# Autodesk Inventor assembly: emsamble caja
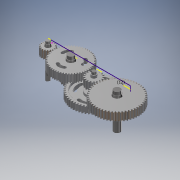
[picture p0: Inventor's stored thumbnail of the model, 180x180]
Saved by Autodesk Inventor 2018 (Build 220112000, 112)
## iProperties
Created: 2017-08-31
Part Number: emsamble caja
Material: Genérico
Document SubType Name: Assembly
Designer: Alumno
Author: Alumno
## Documents named in this file (14)
- D:\Documents\Desktop\proyecto caja reductora-II\emsamble caja.iam
- D:\Documents\Desktop\proyecto caja reductora-II\EJE 2 (30 mm y 15 mm).iam
- D:\Documents\Desktop\proyecto caja reductora-II\TREN 1\Design Accelerator\Engranaje recto12.ipt
- D:\Documents\Desktop\proyecto caja reductora-II\TREN 1\Design Accelerator\Engranaje recto22.ipt
- D:\Documents\Desktop\proyecto caja reductora-II\TREN 2\Design Accelerator\Engranaje recto11.ipt
- D:\Documents\Desktop\proyecto caja reductora-II\TREN 2\Design Accelerator\Engranaje recto21.ipt
- D:\Documents\Desktop\proyecto caja reductora-II\TREN 3\Design Accelerator\Engranaje recto11.ipt
- D:\Documents\Desktop\proyecto caja reductora-II\TREN 3\Design Accelerator\Engranaje recto21.ipt
- D:\Documents\Desktop\proyecto caja reductora-II\EJE 3 (30-45).iam
- D:\Documents\Desktop\proyecto caja reductora-II\EJE 4.iam
- D:\Documents\Desktop\proyecto caja reductora-II\Chaveta- Tren 1.ipt
- D:\Documents\Desktop\proyecto caja reductora-II\Chaveta 25.ipt
- D:\Documents\Desktop\proyecto caja reductora-II\EJE 1.iam
- D:\Documents\Desktop\proyecto caja reductora-II\RODAMIENTO 15 D\6002.iam
## Components (14 placed, 9 different names)
1. Engranaje recto1:1 — Coincidencia:1, Ángulo:2, Coincidencia:16
2. Engranaje recto2:1 — Coincidencia:5, Coincidencia:6, Ángulo:2, Coincidencia:17
3. Engranaje recto2:2 — Coincidencia:12, Coincidencia:13, Coincidencia:18
4. Engranaje recto1:3 — Coincidencia:14, Coincidencia:15
5. Engranaje recto2:3 — Coincidencia:22, Coincidencia:23, Coincidencia:24
6. EJE 2 (30 mm y 15 mm):3 [sub-assembly] — Coincidencia:2, Coincidencia:3, Coincidencia:4, Coincidencia:5, Ángulo:1, Ángulo:3, Coincidencia:17, Nivelación:1, Coincidencia:25, Coincidencia:26
7. Engranaje recto1:4 — Coincidencia:25, Coincidencia:26
8. EJE 3 (30-45):1 [sub-assembly] — Coincidencia:9, Coincidencia:10, Coincidencia:11, Coincidencia:12, Coincidencia:14, Coincidencia:15, Ángulo:3, Coincidencia:18, Ángulo:4, Nivelación:2, Nivelación:3
9. EJE 4:1 [sub-assembly] — Coincidencia:19, Coincidencia:20, Coincidencia:21, Coincidencia:22, Coincidencia:24, Ángulo:4, Nivelación:3
10. Chaveta- Tren 1:1 — Coincidencia:2, Coincidencia:3, Coincidencia:4, Coincidencia:6
11. Chaveta- Tren 1:2 — Coincidencia:19, Coincidencia:20, Coincidencia:21, Coincidencia:23
12. Chaveta 25:6 — Coincidencia:9, Coincidencia:10, Coincidencia:11, Coincidencia:13
13. EJE 1:1 [sub-assembly] — Coincidencia:1, Ángulo:1, Coincidencia:16, Nivelación:1, Nivelación:2
14. 6002:5 [sub-assembly]
## Relationships (31: Mate 24, Angle 4, Flush 3)
- Coincidencia:1 [Mate]: Engranaje recto1:1 ↔ EJE 1:1
- Coincidencia:2 [Mate]: EJE 2 (30 mm y 15 mm):3 ↔ Chaveta- Tren 1:1
- Coincidencia:3 [Mate]: EJE 2 (30 mm y 15 mm):3 ↔ Chaveta- Tren 1:1
- Coincidencia:4 [Mate]: EJE 2 (30 mm y 15 mm):3 ↔ Chaveta- Tren 1:1
- Coincidencia:5 [Mate]: Engranaje recto2:1 ↔ EJE 2 (30 mm y 15 mm):3
- Coincidencia:6 [Mate]: Engranaje recto2:1 ↔ Chaveta- Tren 1:1
- Ángulo:1 [Angle] (0 deg): EJE 2 (30 mm y 15 mm):3 ↔ EJE 1:1
- Ángulo:2 [Angle] (0 deg): Engranaje recto1:1 ↔ Engranaje recto2:1
- Coincidencia:9 [Mate]: EJE 3 (30-45):1 ↔ Chaveta 25:6
- Coincidencia:10 [Mate]: EJE 3 (30-45):1 ↔ Chaveta 25:6
- Coincidencia:11 [Mate]: EJE 3 (30-45):1 ↔ Chaveta 25:6
- Coincidencia:12 [Mate]: Engranaje recto2:2 ↔ EJE 3 (30-45):1
- Coincidencia:13 [Mate]: Engranaje recto2:2 ↔ Chaveta 25:6
- Coincidencia:14 [Mate]: Engranaje recto1:3 ↔ EJE 3 (30-45):1
- Coincidencia:15 [Mate]: Engranaje recto1:3 ↔ EJE 3 (30-45):1
- Ángulo:3 [Angle] (0 deg): EJE 2 (30 mm y 15 mm):3 ↔ EJE 3 (30-45):1
- Coincidencia:16 [Mate]: Engranaje recto1:1 ↔ EJE 1:1
- Coincidencia:17 [Mate]: Engranaje recto2:1 ↔ EJE 2 (30 mm y 15 mm):3
- Coincidencia:18 [Mate]: Engranaje recto2:2 ↔ EJE 3 (30-45):1
- Coincidencia:19 [Mate]: EJE 4:1 ↔ Chaveta- Tren 1:2
- Coincidencia:20 [Mate]: EJE 4:1 ↔ Chaveta- Tren 1:2
- Coincidencia:21 [Mate]: EJE 4:1 ↔ Chaveta- Tren 1:2
- Coincidencia:22 [Mate]: Engranaje recto2:3 ↔ EJE 4:1
- Coincidencia:23 [Mate]: Engranaje recto2:3 ↔ Chaveta- Tren 1:2
- Coincidencia:24 [Mate]: Engranaje recto2:3 ↔ EJE 4:1
- Ángulo:4 [Angle] (0 deg): EJE 3 (30-45):1 ↔ EJE 4:1
- Nivelación:1 [Flush]: EJE 2 (30 mm y 15 mm):3 ↔ EJE 1:1
- Nivelación:2 [Flush]: EJE 3 (30-45):1 ↔ EJE 1:1
- Nivelación:3 [Flush]: EJE 3 (30-45):1 ↔ EJE 4:1
- Coincidencia:25 [Mate]: EJE 2 (30 mm y 15 mm):3 ↔ Engranaje recto1:4
- Coincidencia:26 [Mate]: EJE 2 (30 mm y 15 mm):3 ↔ Engranaje recto1:4
